# Autodesk Inventor assembly: 042-DXP(F,D-166-3)
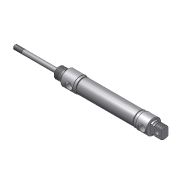
[picture p0: Inventor's stored thumbnail of the model, 180x180]
Saved by Autodesk Inventor 2012 (Build 160160000, 160)
## iProperties
Category: PARTsolutions
Created: 2013-01-22
Part Number: 042-DXP(F,D-166-3)
Catalog Web Link: www.cadenas.de
Description: Original Line Standard Air Cylinders -
Document SubType Name: Assembly
Designer: PARTsolutions
NB: 042-DXP(F,D-166-3)
NN: Original Line Standard Air Cylinders
NBSYN: $PNC.
LINA: 042-DXP
PSOL_MULTISOLIDPART: 0.0
PN: 042-DXP
PNC: 042-DXP(F,D-166-3)
PNA: (D-166-3)
DASH: -
BORE1: 0.75000000
BORE: 3/4" (04)
BOREPN: 04
STROKE: 2.000
STROKEALG: [0.011:50/0.001]
STROKE1: 2.000
ACTING: D
ACTINGALG: '' , 'Single Acting (SA)' , 'R' , 'Reverse Single Acting (SA)' , 'D' , 'Double Acting (SA)'
ACTINGPN: D
MNT: XP
MNTALG: '' , 'Front Nose Mounting (SA)' , 'P' , 'Rear Pivot Mounting (SA)' , 'XP' , 'Double End or Pivot Mounting (SA)' , 'X' , 'Double End Mounting (SA)' , 'BF' , 'Front Block Mounting (SA)' , 'BR' , 'Rear Block Mounting for Vertical Positioning (SA)' , 'BFT' , 'Front Block Trunnion Mounting (SA)' , 'BRT' , 'Rear Block Trunnion Mounting (SA)'
MNTPN: XP
DERALG: '' , 'N/A'
NRALG: '' , 'N/A'
BMALG: '' , 'N/A'
COALG: '' , 'N/A'
OOALG: '', 'N/A'
VO: Z
VOALG: 'Z' , 'N/A'
MALG: '', 'Without Magnet', 'M', 'With Magnet'
EEL: 0.000
EEMAX: 48.0000
EEALG: '', 'Without Extra Extension', 'EE', 'With Extra Extension'
EELALG: 0
EEPN1: 0.000
KALG: '', 'Standard' , 'K' , 'Ports Rotated 90deg K'
QALG: '' , 'N/A'
YALG: '' , 'Without Pivot Bushing' , 'Y' , 'With Pivot Bushing'
FALG: '', 'Non-Coated (Standard)', 'F', 'Molycoated'
TALG: '' , 'Standard -20° to 200°F (-29° to 95°C)' , 'N' , 'Low Temperature' , 'V' , 'High Temperature'
BALG: '', 'W/out Bumpers' , 'B' , 'W/ Bumpers'
HALG: '', 'N/A'
SERALG: '' , 'Without Spring Extend/Return' , 'JS' , 'With Spring Return' , 'JR' , 'With Spring Extend'
SRALG: '' , 'Standard Stainless Steel'
SRCON: 0
WALG: '' , 'Without Wiper' , 'W' , 'With Wiper'
EALG: '' , 'Standard Seals/Lube' , 'E' , 'Non-Lube Seals/Lube'
HLALG: '' , 'Without Low Pressure Hydraulic' , 'HL' , 'With Low Pressure Hydraulic'
STALG: '' , 'N/A'
STPT1ALG: '' , 'N/A'
STPT2ALG: '' , 'N/A'
STPT3ALG: '' , 'N/A'
STPT4ALG: '' , 'N/A'
MBALG: '' , 'Without Mounting Bracket' , 'F,D-129' , 'D-129 (front)'  , 'R,D-129' , 'D-129 (rear)' , '2x,D-129' , 'D-129 (front & rear)'
MBPNALL: D-129
MBPNALLREAR: D-129
PBALG: '' , 'Without Pivot Bracket' , 'D-13498-A' , 'D-13498-A'
PBPNALL: D-13498-A
PRC: F,D-166-3
PRCALG: '' , 'W/out Pivot Rod Clevis' , 'F,D-166-3' , 'D-166-3 (front)'
PRCPN: (F,D-166-3)
PRCPNALL: D-166-3
TBALG: '' , 'N/A'
MNALG: '' , 'N/A'
TLEN: 3.2555
FRAC: 8.7500
RGDACCON: R
RHCON: P
RHCON1: P
RHCONON: 1
FNUTCON: 1
RNUTCON: 1
FNUTPN: D-9
RNUTPN: D-9
FNUTTRANS: 0.0000
RNUTTRANS: 0.0000
VHOLECON: 0
A1: 1.5940
A1N: 0.8750
A1P: 1.5940
A1B: 1.5940
A4: 0.2525
A4N: 0.3130
A4P: 0.2525
A5: 0.0300
A1H: 1.594
A1NH: 0.5310
A1PH: 1.5940
A1BH: 1.0940
A1SH: 1.2190
A2H: 0.2190
A2NH: 0.2190
LENGTH: 3.7500
LENGTH1: 3.7500
LENGTH2: 3.8100
MUL: 2.0000
MUL11: 2.0000
MUL22: 5.380
MUL33: 3.3800
MUL2: 2.0000
MUL211: 2.0000
MUL222: 2.6900
MUL233: 1.6900
SSS: 4.0000
RGLEN: 1.3715
RHLEN: 1.1230
SSS1: 3.0000
A13: 1.3120
DIF: 0.0000
G5: 0.6250
ON: 0
SSADD: 0.0000
BADD: 0.0000
MADD: 0.0000
NVADD: 0.0000
TRACKL: 2.9655
TRACKCON: D-74168
TRIMCON: 0
TRIMCON1: 0
PINCON: D-51
FSPACE: 0.6926
SPACE: 0.0643
TEXT: 0.1125
S1: 1.0000
D1: 0.8325
D1N: 0.8050
D1B: 0.8625
D1P: 0.8325
FA: 0.940
RA: 0.9400
PPATH: standard_air_cylinder_asmtpl.prj
MATALGHTML: <b>Standard Original Line:</b><dl><dt>Rod:</dt><dd>- Stainless Steel</dd><dd>&nbsp;&nbsp;(5/16 ? 9/16 Bores)</dd><dd>- High Strength Carbon Steel</dd><dd>&nbsp;&nbsp;(3/4 ? 3 Bore)</dd><dd>- Stainless Steel</dd><dd>&nbsp;&nbsp;(?X? style DXP/DX/DXDE?)</dd><dt>Bearings:</dt><dd>- Sintered Bronze</dd><dt>Body:</dt><dd>- 304 Stainless Steel</dd><dt>End Caps:</dt><dd>- Aluminum</dd><dt>Seals:</dt><dd>- Buna N</dd></dl>
ASSCFGPRA: 04DXP
PRCPNA: (D-166-3)
ASSOPTACC: STPT4
A: 5.75
HADD: 0.0000
WFL: 0.250
QADD: 0.000
QADD1: 0.440
TEST: 2.0000
STDNUTF: 1
STDNUTR: 1
KT: DUMMY
CreationOption_UseAsmMates: false
SUPPLIER: Bimba
ARTICLENO: 042-DXP(F,D-166-3)
BOMINFO: 042-DXP
CREATOR: CADENAS GmbH
PSOL_IDENT_0: {\\10.0.0.242\data_v9\23d-libs\bimba\bimba\bimba_imperial\bimba_full_line\original_line_cylinders\st
PSOL_IDENT_1: andard_air_cylinders\standard_air_cylinder_asmtab.prj},316 {VTYP=3D},{STYP=ASSTAB},{NB=042-DXP(F,D-1
PSOL_IDENT_2: 66-3)},{LINA=042-DXP},{NN=Original Line Standard Air Cylinders},{DATE=06.09.2012 11:26:56},{GEOMDATE
PSOL_IDENT_3: =06.09.2012},{VERSION=},{LINEID=50},{LINESUBID=-1},{WBVAR=STROKE,ACTING,MNT,DER,NR,BM,CO,OO,VO,M,EE,
PSOL_IDENT_4: EEL,K,Q,Y,G,T,B,H,SER,SR,NT,W,HL,STPT1,STPT2,STPT3,STPT4,MB,PB,PRC,TB,MN}  {NB=042-DXP(F,D-166-3)},{
PSOL_IDENT_5: LINA=042-DXP},{KT=DUMMY},{PN=042-DXP},{PNC=042-DXP(F,D-166-3)},{PNA=(D-166-3)},{DASH=-},{BORE1=0.750
PSOL_IDENT_6: 00000},{BORE=3/4\" (04)},{BOREPN=04},{STROKE=2.000},{STROKEALG=[0.011:50/0.001]},{STROKE1=2.000},{AC
PSOL_IDENT_7: TING=D},{ACTINGALG= '' , 'Single Acting (SA)' , 'R' , 'Reverse Single Acting (SA)' , 'D' , 'Double A
PSOL_IDENT_8: cting (SA)' },{ACTINGPN=D},{MNT=XP},{MNTALG= '' , 'Front Nose Mounting (SA)' , 'P' , 'Rear Pivot Mou
PSOL_IDENT_9: nting (SA)' , 'XP' , 'Double End or Pivot Mounting (SA)' , 'X' , 'Double End Mounting (SA)' , 'BF' ,
PSOL_IDENT_10: 'Front Block Mounting (SA)' , 'BR' , 'Rear Block Mounting for Vertical Positioning (SA)' , 'BFT' ,
PSOL_IDENT_11: 'Front Block Trunnion Mounting (SA)' , 'BRT' , 'Rear Block Trunnion Mounting (SA)' },{TYPE=},{MNTPN=
PSOL_IDENT_12: XP},{DER=},{DERALG= '' , 'N/A' },{NR=},{NRALG= '' , 'N/A' },{NRPN=},{BM=},{BMALG= '' , 'N/A' },{BMPN
PSOL_IDENT_13: =},{CO=},{COALG= '' , 'N/A' },{OO=},{OOALG= '', 'N/A' },{OOPN=},{VO=Z},{VOALG= 'Z' , 'N/A' },{VOPN=}
PSOL_IDENT_14: ,{OOVOPN=},{M=},{MALG= '', 'Without Magnet', 'M', 'With Magnet' },{EE=},{EEL=0.000},{EEMAX=48.0000},
PSOL_IDENT_15: {EEALG= '', 'Without Extra Extension', 'EE', 'With Extra Extension' },{EELALG=0},{EEPN=},{EEPN1=0.00
PSOL_IDENT_16: 0},{K=},{KALG= '', 'Standard' , 'K' , 'Ports Rotated 90deg K' },{KPN=},{Q=},{QALG= '' , 'N/A' },{QPN
PSOL_IDENT_17: =},{Y=},{YALG= '' , 'Without Pivot Bushing' , 'Y' , 'With Pivot Bushing' },{YPN=},{YCON=},{F=},{FALG
PSOL_IDENT_18: = '', 'Non-Coated (Standard)', 'F', 'Molycoated' },{FPN=},{G=},{GPN=},{GPN99=},{T=},{TALG= '' , 'Sta
PSOL_IDENT_19: ndard -20° to 200°F (-29° to 95°C)' , 'N' , 'Low Temperature' , 'V' , 'High Temperature' },{NPN=},{V
PSOL_IDENT_20: PN=},{B=},{BALG= '', 'W/out Bumpers' , 'B' , 'W/ Bumpers' },{BPN=},{H=},{HALG= '', 'N/A' },{HPN=},{S
PSOL_IDENT_21: ER=},{SERALG= '' , 'Without Spring Extend/Return' , 'JS' , 'With Spring Return' , 'JR' , 'With Sprin
PSOL_IDENT_22: g Extend' },{SR=},{SRALG= '' , 'Standard Stainless Steel' },{SRPN=},{SRCON=0},{NT=},{NTPN=},{W=},{WA
PSOL_IDENT_23: LG= '' , 'Without Wiper' , 'W' , 'With Wiper' },{WPN=},{E=},{EALG= '' , 'Standard Seals/Lube' , 'E'
PSOL_IDENT_24: , 'Non-Lube Seals/Lube' },{EPN=},{HL=},{HLALG= '' , 'Without Low Pressure Hydraulic' , 'HL' , 'With
PSOL_IDENT_25: Low Pressure Hydraulic' },{ST=},{STALG= '' , 'N/A' },{STPT1=},{STPT1ALG= '' , 'N/A' },{STPT2=},{STPT
PSOL_IDENT_26: 2ALG= '' , 'N/A' },{STPT3=},{STPT3ALG= '' , 'N/A' },{STPT4=},{STPT4ALG= '' , 'N/A' },{STPN=},{MB=},{
PSOL_IDENT_27: MBALG= '' , 'Without Mounting Bracket' , 'F,D-129' , 'D-129 (front)'  , 'R,D-129' , 'D-129 (rear)' ,
PSOL_IDENT_28: '2x,D-129' , 'D-129 (front & rear)'},{MBPN=},{MBPNALL=D-129},{MBPNALLREAR=D-129},{PB=},{PBALG= '' ,
PSOL_IDENT_29: 'Without Pivot Bracket' , 'D-13498-A' , 'D-13498-A' },{PBPN=},{PBPNALL=D-13498-A},{PRC=F,D-166-3},{
PSOL_IDENT_30: PRCALG= '' , 'W/out Pivot Rod Clevis' , 'F,D-166-3' , 'D-166-3 (front)' },{PRCPN=(F,D-166-3)},{PRCPN
PSOL_IDENT_31: ALL=D-166-3},{TB=},{TBALG= '' , 'N/A' },{TBPN=},{TBPNALL=},{MN=},{MNALG= '' , 'N/A' },{MNPN=},{MNCON
PSOL_IDENT_32: F=},{MNCONR=},{TLEN=3.2555},{FRAC=8.7500},{RGCON=},{RGDACCON=R},{RHCON=P},{RHCON1=P},{RHCONON=1},{RH
PSOL_IDENT_33: ACCON=},{FNUTCON=1},{RNUTCON=1},{FNUTPN=D-9},{RNUTPN=D-9},{FNUTTRANS=0.0000},{RNUTTRANS=0.0000},{VHO
PSOL_IDENT_34: LECON=0},{A1=1.5940},{A1N=0.8750},{A1P=1.5940},{A1B=1.5940},{A4=0.2525},{A4N=0.3130},{A4P=0.2525},{A
PSOL_IDENT_35: 5=0.0300},{A1H=1.594},{A1NH=0.5310},{A1PH=1.5940},{A1BH=1.0940},{A1SH=1.2190},{A2H=0.2190},{A2NH=0.2
PSOL_IDENT_36: 190},{LENGTH=3.7500},{LENGTH1=3.7500},{LENGTH2=3.8100},{MUL=2.0000},{MUL11=2.0000},{MUL22=5.38},{MUL
PSOL_IDENT_37: 33=3.3800},{MUL2=2.0000},{MUL211=2.0000},{MUL222=2.6900},{MUL233=1.6900},{SSS=4.0000},{RGLEN=1.3715}
PSOL_IDENT_38: ,{RHLEN=1.1230},{SSS1=3.0000},{A13=1.3120},{DIF=0.0000},{G5=0.6250},{ON=0},{SSADD=0.0000},{BADD=0.00
PSOL_IDENT_39: 00},{MADD=0.0000},{NVADD=0.0000},{TRACKL=2.9655},{TRACKCON=D-74168},{TRIMCON=0},{TRIMCON1=0},{PINCON
PSOL_IDENT_40: =D-51},{FSPACE=0.6926},{SPACE=0.0643},{TEXT=0.1125},{S1=1.0000},{D1=0.8325},{D1N=0.8050},{D1B=0.8625
PSOL_IDENT_41: },{D1P=0.8325},{FA=0.940},{RA=0.9400},{PPATH=standard_air_cylinder_asmtpl.prj},{MATALGHTML=<b>Standa
PSOL_IDENT_42: rd Original Line:</b><dl><dt>Rod:</dt><dd>- Stainless Steel</dd><dd>&nbsp;&nbsp;(5/16 ? 9/16 Bores)<
PSOL_IDENT_43: /dd><dd>- High Strength Carbon Steel</dd><dd>&nbsp;&nbsp;(3/4 ? 3 Bore)</dd><dd>- Stainless Steel</d
PSOL_IDENT_44: d><dd>&nbsp;&nbsp;(?X? style DXP/DX/DXDE?)</dd><dt>Bearings:</dt><dd>- Sintered Bronze</dd><dt>Body:
PSOL_IDENT_45: </dt><dd>- 304 Stainless Steel</dd><dt>End Caps:</dt><dd>- Aluminum</dd><dt>Seals:</dt><dd>- Buna N<
PSOL_IDENT_46: /dd></dl>},{ASSCFGPRA=04DXP},{MBPNA=},{MNPNA=},{PRCPNA=(D-166-3)},{ASSOPTACC=STPT4},{A=5.75},{HADD=0
PSOL_IDENT_47: .0000},{WFL=0.25},{QADD=0.000},{QADD1=0.440},{TEST=2.0000},{MNTB=},{STDNUTF=1},{STDNUTR=1}
Title: 042-DXP
Author: Cadenas PARTsolutions
## Documents named in this file (6)
- Z:\UserData\Documents\Inventor\team1885frc\Pneumatics\042-DXP_2inStrokex075Bore\042_DXP_F_D_166_3_.iam
- Z:\UserData\Documents\Inventor\team1885frc\Pneumatics\042-DXP_2inStrokex075Bore\04R000_rod_guide.ipt
- Z:\UserData\Documents\Inventor\team1885frc\Pneumatics\042-DXP_2inStrokex075Bore\042_DXP0_rod.ipt
- Z:\UserData\Documents\Inventor\team1885frc\Pneumatics\042-DXP_2inStrokex075Bore\D_166_3_dummy.ipt
- Z:\UserData\Documents\Inventor\team1885frc\Pneumatics\042-DXP_2inStrokex075Bore\04R_3_25550.ipt
- Z:\UserData\Documents\Inventor\team1885frc\Pneumatics\042-DXP_2inStrokex075Bore\04P0000_rear_head.ipt
## Components (5 placed, 5 different names)
1. 04R000_rod_guide:1 — Mate:1
2. D-166-3-dummy:1
3. 04R-3.25550:1
4. 04P0000_rear_head:1 — Mate:2
5. 042-DXP0_rod:1 — Mate:1, Mate:2
## Relationships (2: Mate 2)
- Mate:1: 04R000_rod_guide:1 ↔ 042-DXP0_rod:1
- Mate:2: 04P0000_rear_head:1 ↔ 042-DXP0_rod:1
